# Autodesk Inventor assembly: Optical Shaft (Quadrature) Encoder
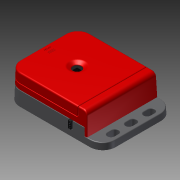
[picture p0: Inventor's stored thumbnail of the model, 180x180]
Saved by Autodesk Inventor 2014 SP1 (Build 180222100, 222)
## iProperties
Created: 2010-04-29
Part Number: Optical Shaft (Quadrature) Encoder
Document SubType Name: Assembly
Designer: Jordan
Mass: 35.38 g
Surface Area: 286.622 cm^2
Volume: 20.9134 cm^3
Translation Standard: STEP AP203
FileName: Optical Shaft (Quadrature) Encoder.iam
PreProcessor: SolidWorks 2006052
PostProcessor: Build: 239, Release: 2011 RTM - Date: Wed 02/17/2010
Sent Units: inch
Uncertainty: 1e-05
Author: Jordan
## Documents named in this file (6)
- C:\Users\Ryan\Desktop\sw\lib\Super Sonic Sparks VEX CAD Library\Motors & Sensors\Optical Shaft (Quadrature) Encoder.iam
- C:\Users\Ryan\Desktop\sw\lib\Super Sonic Sparks VEX CAD Library\Motors & Sensors\Optical Shaft (Quadrature) Encoder-Parts\Top.ipt
- C:\Users\Ryan\Desktop\sw\lib\Super Sonic Sparks VEX CAD Library\Motors & Sensors\Optical Shaft (Quadrature) Encoder-Parts\Wheel.ipt
- C:\Users\Ryan\Desktop\sw\lib\Super Sonic Sparks VEX CAD Library\Motors & Sensors\Optical Shaft (Quadrature) Encoder-Parts\Wire Sleeve.ipt
- C:\Users\Ryan\Desktop\sw\lib\Super Sonic Sparks VEX CAD Library\Motors & Sensors\Optical Shaft (Quadrature) Encoder-Parts\Middle.ipt
- C:\Users\Ryan\Desktop\sw\lib\Super Sonic Sparks VEX CAD Library\Motors & Sensors\Optical Shaft (Quadrature) Encoder-Parts\Bottom.ipt
## Components (5 placed, 5 different names)
1. Top:1
2. Wheel:1
3. Wire Sleeve:1 — Angle:1
4. Middle:1
5. Bottom:1 — Mate:1, Mate:2, Mate:3, Mate:4
## Relationships (8: Mate 7, Angle 1)
- Mate:1 (2.25 mm): Bottom:1
- Mate:2 (2.25 mm): Bottom:1
- Mate:3 (25 mm): Bottom:1
- Mate:4 (25 mm): Bottom:1
- Mate:5
- Mate:6
- Mate:7
- Angle:1 (0 deg): Wire Sleeve:1
